# Autodesk Inventor assembly: total_montaj
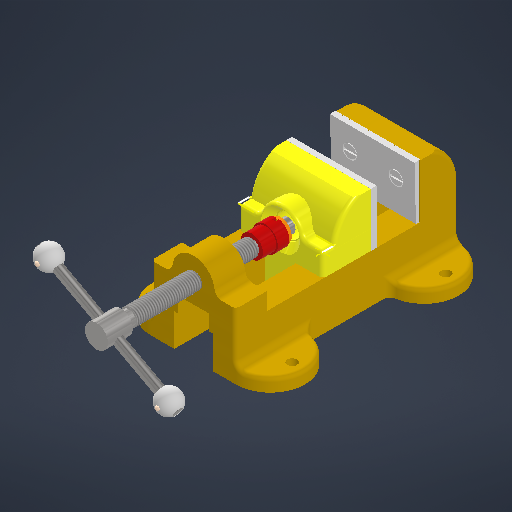
[picture p0: Inventor's stored thumbnail of the model, 512x512]
Saved by Autodesk Inventor 2025.4 (Build 294407000, 407)
## iProperties
Created: 2026-06-20
Part Number: total_montaj
Document SubType Name: Weldment
Designer: yigithan
Weld Material: Welded Aluminum-6061
Author: yigithan
## Documents named in this file (6)
- C:\Users\yigithan\Desktop\mengene\total_montaj.iam
- C:\Users\yigithan\Desktop\mengene\alt_plaka.ipt
- C:\Users\yigithan\Desktop\mengene\haraketli_palaka.ipt
- C:\Users\yigithan\Desktop\mengene\plaka.ipt
- C:\Users\yigithan\Documents\Inventor\Content Center Files\R2025\en-US\AS 1427(03)\AS 1427 - M6 x 16(1).ipt
- C:\Users\yigithan\Desktop\mengene\vida_mili_montaj.iam
## Components (9 placed, 5 different names)
1. alt_plaka:1 — Mate:1, Mate:2, Mate:3, Mate:4, Mate:5, Mate:8
2. haraketli_palaka:1 — Mate:1, Mate:2, Mate:6, Mate:7, Mate:9
3. plaka:1 — Mate:6, Mate:7, Insert:1, Insert:2
4. plaka:2 — Mate:3, Mate:4, Mate:5, Insert:3, Insert:4
5. AS 1427 - Metric M6 x 16:1 — Insert:3
6. AS 1427 - Metric M6 x 16:2 — Insert:4
7. AS 1427 - Metric M6 x 16:3 — Insert:1
8. AS 1427 - Metric M6 x 16:4 — Insert:2
9. vida_mili_montaj:1 [sub-assembly] — Mate:8, Mate:9
## Relationships (13: Mate 9, Insert 4)
- Mate:1: alt_plaka:1 ↔ haraketli_palaka:1
- Mate:2: alt_plaka:1 ↔ haraketli_palaka:1
- Mate:3: alt_plaka:1 ↔ plaka:2
- Mate:4: alt_plaka:1 ↔ plaka:2
- Mate:5: alt_plaka:1 ↔ plaka:2
- Mate:6: haraketli_palaka:1 ↔ plaka:1
- Mate:7: haraketli_palaka:1 ↔ plaka:1
- Insert:1: plaka:1 ↔ AS 1427 - Metric M6 x 16:3
- Insert:2: plaka:1 ↔ AS 1427 - Metric M6 x 16:4
- Insert:3: plaka:2 ↔ AS 1427 - Metric M6 x 16:1
- Insert:4: plaka:2 ↔ AS 1427 - Metric M6 x 16:2
- Mate:8: alt_plaka:1 ↔ vida_mili_montaj:1
- Mate:9: haraketli_palaka:1 ↔ vida_mili_montaj:1
